# Autodesk Inventor assembly: upper_leg_link
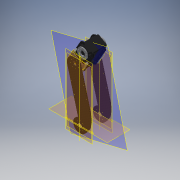
[picture p0: Inventor's stored thumbnail of the model, 180x180]
Saved by Autodesk Inventor 2018 (Build 220112000, 112)
## iProperties
Created: 2018-11-30
Part Number: upper_leg_link
Document SubType Name: Assembly
Designer: bitbots
Author: bitbots
## Documents named in this file (4)
- C:\Users\jaspe\bitbots_hardware\wolfgang\assembly\legs\upper_leg_link.iam
- C:\Users\jaspe\bitbots_hardware\wolfgang\assembly\legs\upper_leg_MIR.ipt
- C:\Users\jaspe\bitbots_hardware\wolfgang\assembly\motors\MX106\MX-106_with_bearing_MIR.iam
- C:\Users\jaspe\bitbots_hardware\wolfgang\assembly\legs\knee_connector_MIR.ipt
## Components (5 placed, 3 different names)
1. upper_leg_MIR:1 — Symmetry:1, Mate:13, Mate:14, Mate:16
2. upper_leg_MIR:2 — Symmetry:1, Mate:15
3. MX-106_with_bearing_MIR:1 [sub-assembly] — Mate:17
4. knee_connector_MIR:1
5. knee_connector_MIR:2 — Mate:13
## Relationships (20: Mate 17, Flush 2, Symmetry 1)
- [Mate] (0.65 mm): upper_leg_MIR:2 ↔ knee_connector_MIR:1
- [Mate]: upper_leg_MIR:2 ↔ knee_connector_MIR:1
- [Mate]: upper_leg_MIR:2 ↔ knee_connector_MIR:1
- [Mate]: MX-106_with_bearing_MIR:1 ↔ knee_connector_MIR:1
- [Mate]: MX-106_with_bearing_MIR:1 ↔ knee_connector_MIR:1
- [Mate]: MX-106_with_bearing_MIR:1 ↔ knee_connector_MIR:1
- [Mate]: upper_leg_MIR:1 ↔ knee_connector_MIR:2
- [Mate]: upper_leg_MIR:1 ↔ knee_connector_MIR:2
- [Mate]: MX-106_with_bearing_MIR:1 ↔ knee_connector_MIR:2
- [Mate]: MX-106_with_bearing_MIR:1 ↔ knee_connector_MIR:2
- [Mate]: MX-106_with_bearing_MIR:1 ↔ knee_connector_MIR:2
- [Mate] (0.65 mm): upper_leg_MIR:2 ↔ knee_connector_MIR:1
- Symmetry:1: upper_leg_MIR:1 ↔ upper_leg_MIR:2
- Flush:1
- Mate:13: upper_leg_MIR:1 ↔ knee_connector_MIR:2
- Mate:14: upper_leg_MIR:1
- Mate:15: upper_leg_MIR:2
- Flush:2
- Mate:16: upper_leg_MIR:1
- Mate:17: MX-106_with_bearing_MIR:1
